# Autodesk Inventor assembly: boil
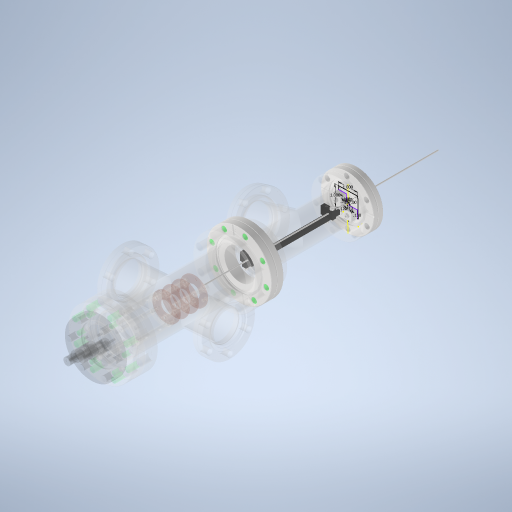
[picture p0: Inventor's stored thumbnail of the model, 512x512]
Saved by Autodesk Inventor 2024 (Build 280153000, 153)
## iProperties
Created: 2023-04-15
Part Number: boil
Document SubType Name: Assembly
Designer: Fujitsu
Author: Fujitsu
## Documents named in this file (12)
- C:\Users\Fujitsu\Raad\BaTag\boil.iam
- C:\Users\Fujitsu\Raad\BaTag\dff275x000\dff275x000-drilled.ipt
- C:\Users\Fujitsu\Raad\BaTag\capillary.ipt
- C:\Users\Fujitsu\Raad\BaTag\clamp2.ipt
- C:\Users\Fujitsu\Raad\BaTag\rod1.ipt
- C:\Users\Fujitsu\Raad\BaTag\cWasher.ipt
- C:\Users\Fujitsu\Raad\BaTag\tab.ipt
- C:\Users\Fujitsu\Raad\BaTag\cScrew.ipt
- C:\Users\Fujitsu\Raad\BaTag\ssVScrew.ipt
- C:\Users\Fujitsu\Raad\BaTag\tee.iam
- C:\Users\Fujitsu\Raad\BaTag\zwj.ipt
- C:\Users\Fujitsu\Raad\BaTag\detector_chamber3\detector_chamber3.iam
## Components (17 placed, 11 different names)
1. dff275x000-drilled:1 — Mate:1, Angle:1, Angle:2, Angle:3, Angle:4, Mate:10, Mate:17
2. capillary:1 — Mate:1, Angle:1, Mate:2, Mate:3, Mate:16, Mate:18, Mate:20
3. clamp2:1 — Mate:2, Angle:2, Mate:4, Mate:12, Mate:13, Mate:15
4. clamp2:2 — Mate:3, Angle:3, Mate:5, Insert:4
5. rod1:1 — Mate:4, Mate:5, Mate:6, Mate:7, Insert:3, Mate:12, Mate:13, Mate:14
6. cWasher:1 — Mate:6, Mate:7, Mate:8, Mate:9
7. tab:1 — Mate:8, Mate:9, Angle:4, Mate:10, Insert:1, Mate:11, Insert:2, Insert:5
8. cScrew:1 — Insert:1
9. ssVScrew:1 — Mate:11, Insert:5
10. ssVScrew:2 — Insert:2
11. ssVScrew:3 — Insert:3
12. ssVScrew:4 — Mate:14
13. ssVScrew:5 — Mate:15
14. ssVScrew:6 — Insert:4
15. tee:1 [sub-assembly] — Mate:16, Mate:17, Mate:19
16. zwj:1 — Mate:18, Mate:19, Mate:21
17. detector_chamber3:1 [sub-assembly] — Mate:20, Mate:21
## Relationships (30: Mate 21, Insert 5, Angle 4)
- Mate:1: dff275x000-drilled:1 ↔ capillary:1
- Angle:1 (90 deg): dff275x000-drilled:1 ↔ capillary:1
- Mate:2: capillary:1 ↔ clamp2:1
- Mate:3: capillary:1 ↔ clamp2:2
- Angle:2 (0 deg): dff275x000-drilled:1 ↔ clamp2:1
- Angle:3 (0 deg): dff275x000-drilled:1 ↔ clamp2:2
- Mate:4: clamp2:1 ↔ rod1:1
- Mate:5: clamp2:2 ↔ rod1:1
- Mate:6: rod1:1 ↔ cWasher:1
- Mate:7: rod1:1 ↔ cWasher:1
- Mate:8: cWasher:1 ↔ tab:1
- Mate:9: cWasher:1 ↔ tab:1
- Angle:4 (180 deg): dff275x000-drilled:1 ↔ tab:1
- Mate:10: dff275x000-drilled:1 ↔ tab:1
- Insert:1: tab:1 ↔ cScrew:1
- Mate:11: tab:1 ↔ ssVScrew:1
- Insert:2: tab:1 ↔ ssVScrew:2
- Insert:3: rod1:1 ↔ ssVScrew:3
- Mate:12: clamp2:1 ↔ rod1:1
- Mate:13: clamp2:1 ↔ rod1:1
- Mate:14: rod1:1 ↔ ssVScrew:4
- Mate:15: clamp2:1 ↔ ssVScrew:5
- Insert:4: clamp2:2 ↔ ssVScrew:6
- Mate:16: capillary:1 ↔ tee:1
- Mate:17: dff275x000-drilled:1 ↔ tee:1
- Insert:5: tab:1 ↔ ssVScrew:1
- Mate:18: capillary:1 ↔ zwj:1
- Mate:19: tee:1 ↔ zwj:1
- Mate:20: capillary:1 ↔ detector_chamber3:1
- Mate:21: zwj:1 ↔ detector_chamber3:1
